# Autodesk Inventor assembly: Guss+erweitertes_Innen
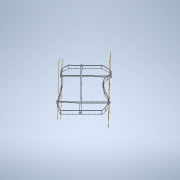
[picture p0: Inventor's stored thumbnail of the model, 180x180]
Saved by Autodesk Inventor 2020.3 (Build 243373000, 373)
## iProperties
Created: 2020-11-14
Part Number: Guss+erweitertes_Innen
Document SubType Name: Assembly
Designer: Mara
Author: Mara
## Documents named in this file (3)
- C:\Users\Mara\Masterarbeit_CAD\Guss+erweitertes_Innen.iam
- C:\Users\Mara\Masterarbeit_CAD\Guss_mit_Halterungsbereich.ipt
- C:\Users\Mara\Masterarbeit_CAD\Innenhalterung_erweitert.ipt
## Components (2 placed, 2 different names)
1. Guss_mit_Halterungsbereich:1 — Mate:1, Mate:2, Mate:3, Mate:4
2. Innenhalterung_erweitert:1 — Mate:1, Mate:2, Mate:3, Mate:4
## Relationships (4: Mate 4)
- Mate:1 (3 mm): Guss_mit_Halterungsbereich:1 ↔ Innenhalterung_erweitert:1
- Mate:2 (0.2 mm): Guss_mit_Halterungsbereich:1 ↔ Innenhalterung_erweitert:1
- Mate:3 (0.2 mm): Guss_mit_Halterungsbereich:1 ↔ Innenhalterung_erweitert:1
- Mate:4 (0.2 mm): Guss_mit_Halterungsbereich:1 ↔ Innenhalterung_erweitert:1
